# Autodesk Inventor assembly: 射出_本体
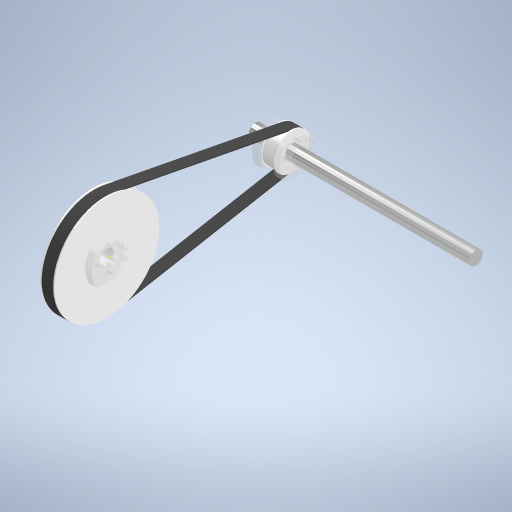
[picture p0: Inventor's stored thumbnail of the model, 512x512]
Saved by Autodesk Inventor 2023 (Build 270158000, 158)
## iProperties
Created: 2022-04-24
Part Number: 射出_本体
Document SubType Name: Assembly
Designer: yuta
Author: yuta
## Documents named in this file (8)
- C:\Users\yuta\Documents\NHK\射出_本体.iam
- C:\Users\yuta\Documents\NHK\type4.ipt
- C:\Users\yuta\Documents\NHK\type3.ipt
- C:\Users\yuta\Documents\NHK\type2.ipt
- C:\Users\yuta\Documents\NHK\射出_軸.ipt
- C:\Users\yuta\Documents\NHK\射出_腕固定.ipt
- C:\Users\yuta\Documents\NHK\射出_腕固定2.ipt
- C:\Users\yuta\Documents\NHK\射出_腕固定3.ipt
## Components (8 placed, 7 different names)
1. type4:1 — メイト:1, メイト:2, メイト:3, メイト:4
2. type3:1 — メイト:1, メイト:2, メイト:10, メイト:11, メイト:12, メイト:13
3. type2:1 — メイト:3, メイト:4, メイト:5, メイト:6, フラッシュ:1, メイト:9
4. 射出_軸:1 — メイト:5, フラッシュ:1, メイト:7, メイト:8
5. 射出_腕固定:1 — メイト:6, メイト:7
6. 射出_腕固定:2 — メイト:8, メイト:9
7. 射出_腕固定2:1 — メイト:10, メイト:11
8. 射出_腕固定3:1 — メイト:12, メイト:13
## Relationships (14: Mate 13, Flush 1)
- メイト:1 [Mate]: type4:1 ↔ type3:1
- メイト:2 [Mate]: type4:1 ↔ type3:1
- メイト:3 [Mate]: type4:1 ↔ type2:1
- メイト:4 [Mate]: type4:1 ↔ type2:1
- メイト:5 [Mate]: type2:1 ↔ 射出_軸:1
- メイト:6 [Mate]: type2:1 ↔ 射出_腕固定:1
- フラッシュ:1 [Flush] (20 mm): type2:1 ↔ 射出_軸:1
- メイト:7 [Mate]: 射出_軸:1 ↔ 射出_腕固定:1
- メイト:8 [Mate]: 射出_軸:1 ↔ 射出_腕固定:2
- メイト:9 [Mate]: type2:1 ↔ 射出_腕固定:2
- メイト:10 [Mate]: type3:1 ↔ 射出_腕固定2:1
- メイト:11 [Mate]: type3:1 ↔ 射出_腕固定2:1
- メイト:12 [Mate]: type3:1 ↔ 射出_腕固定3:1
- メイト:13 [Mate]: type3:1 ↔ 射出_腕固定3:1
